# Autodesk Inventor assembly: Second Case
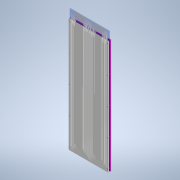
[picture p0: Inventor's stored thumbnail of the model, 180x180]
Saved by Autodesk Inventor 2021 (Build 250183000, 183)
## iProperties
Created: 2022-02-06
Part Number: Second Case
Document SubType Name: Assembly
Designer: tlar613
Author: tlar613
## Documents named in this file (8)
- \\unifiles.uoa.auckland.ac.nz\myhome\Documents\GitHub\2021_SRW_RC_CAR\Magnetics\Final Coil Design\CadModels\SecondCasing\Second Case.iam
- \\unifiles.uoa.auckland.ac.nz\myhome\Documents\GitHub\2021_SRW_RC_CAR\Magnetics\Final Coil Design\CadModels\SecondCasing\Base.ipt
- \\unifiles.uoa.auckland.ac.nz\myhome\Documents\GitHub\2021_SRW_RC_CAR\Magnetics\Final Coil Design\CadModels\SecondCasing\AluminumCasing.ipt
- \\unifiles.uoa.auckland.ac.nz\myhome\Documents\GitHub\2021_SRW_RC_CAR\Magnetics\Final Coil Design\CadModels\SecondCasing\AluminumSheet.ipt
- \\unifiles.uoa.auckland.ac.nz\myhome\Documents\GitHub\2021_SRW_RC_CAR\Magnetics\Final Coil Design\CadModels\SecondCasing\FerriteLayer.ipt
- \\unifiles.uoa.auckland.ac.nz\myhome\Documents\GitHub\2021_SRW_RC_CAR\Magnetics\Final Coil Design\CadModels\SecondCasing\CoilCasing.ipt
- \\unifiles.uoa.auckland.ac.nz\myhome\Documents\GitHub\2021_SRW_RC_CAR\Magnetics\Final Coil Design\CadModels\SecondCasing\FerriteLayer2.ipt
- \\unifiles.uoa.auckland.ac.nz\myhome\Documents\GitHub\2021_SRW_RC_CAR\Magnetics\Final Coil Design\CadModels\SecondCasing\rod.ipt
## Components (16 placed, 7 different names)
1. Base:1 — Mate:1, Mate:2, Flush:13, Flush:14
2. AluminumCasing:1 — Mate:1, Mate:4, Mate:5, Mate:7, Flush:13, Flush:14, Flush:19, Flush:20
3. AluminumSheet:1 — Mate:2, Mate:4, Mate:7
4. FerriteLayer:1 — Mate:5, Mate:8, Flush:16, Flush:20, Flush:21
5. CoilCasing:1 — Mate:9, Flush:18, Flush:19, Insert:1, Insert:2, Insert:3, Insert:4, Insert:5, Insert:6, Insert:7, Insert:8, Insert:9, Insert:10
6. FerriteLayer2:1 — Mate:8, Flush:16, Mate:9, Flush:18, Flush:21
7. rod:1 — Insert:10
8. rod:2 — Insert:9
9. rod:3 — Insert:8
10. rod:4 — Insert:7
11. rod:5 — Insert:6
12. rod:6 — Insert:5
13. rod:7 — Insert:4
14. rod:8 — Insert:3
15. rod:9 — Insert:2
16. rod:10 — Insert:1
## Relationships (24: Insert 10, Mate 7, Flush 7)
- Mate:1: Base:1 ↔ AluminumCasing:1
- Mate:2: Base:1 ↔ AluminumSheet:1
- Mate:4: AluminumCasing:1 ↔ AluminumSheet:1
- Mate:5: AluminumCasing:1 ↔ FerriteLayer:1
- Mate:7: AluminumCasing:1 ↔ AluminumSheet:1
- Flush:13: Base:1 ↔ AluminumCasing:1
- Flush:14: Base:1 ↔ AluminumCasing:1
- Mate:8: FerriteLayer:1 ↔ FerriteLayer2:1
- Flush:16: FerriteLayer:1 ↔ FerriteLayer2:1
- Mate:9: CoilCasing:1 ↔ FerriteLayer2:1
- Flush:18: CoilCasing:1 ↔ FerriteLayer2:1
- Flush:19: AluminumCasing:1 ↔ CoilCasing:1
- Flush:20: AluminumCasing:1 ↔ FerriteLayer:1
- Insert:1: CoilCasing:1 ↔ rod:10
- Insert:2: CoilCasing:1 ↔ rod:9
- Insert:3: CoilCasing:1 ↔ rod:8
- Insert:4: CoilCasing:1 ↔ rod:7
- Insert:5: CoilCasing:1 ↔ rod:6
- Insert:6: CoilCasing:1 ↔ rod:5
- Insert:7: CoilCasing:1 ↔ rod:4
- Insert:8: CoilCasing:1 ↔ rod:3
- Insert:9: CoilCasing:1 ↔ rod:2
- Insert:10: CoilCasing:1 ↔ rod:1
- Flush:21: FerriteLayer:1 ↔ FerriteLayer2:1
